# Autodesk Inventor assembly: SolarPanel
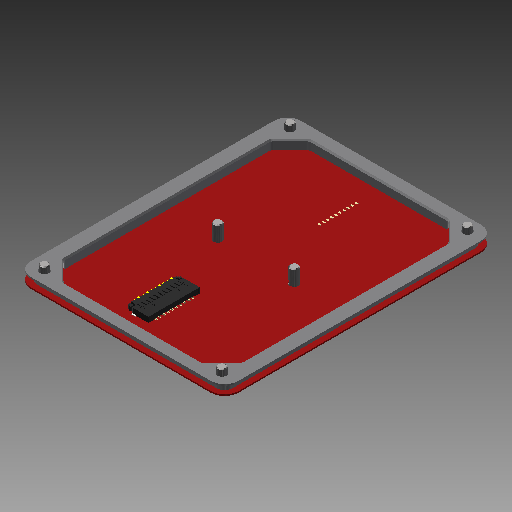
[picture p0: Inventor's stored thumbnail of the model, 512x512]
Saved by Autodesk Inventor 2018 (Build 220112000, 112)
## iProperties
Created: 2018-05-13
Part Number: SolarPanel
Document SubType Name: Assembly
Designer: Bradley
Mass: 16.4819 g
Surface Area: 334.424 cm^2
Volume: 10.2894 cm^3
Density: 1.60184 g/cm^3
Author: Bradley
## Documents named in this file (7)
- D:\Users\Bradley\Documents\CougsInSpace\CougSat1-Hardware\CougSat1-PowerBoard\CADModel\Native\SolarPanel+Y.iam
- D:\Users\Bradley\Documents\CougsInSpace\CougSat1-Hardware\CougSat1-PowerBoard\CADModel\Native\SolarPanel_PCB.ipt
- D:\Users\Bradley\Documents\CougsInSpace\CougSat1-Hardware\CougSat1-PowerBoard\CADModel\Native\SolarPanel_CoilForm.ipt
- D:\Users\Bradley\Documents\CougsInSpace\Resources\ComponentModels\Electronics\SolarCell_UTJ.ipt
- D:\Users\Bradley\Documents\CougsInSpace\Resources\ComponentModels\Fasteners\Bolt_M3x0.35_6mm_BH.ipt
- D:\Users\Bradley\Documents\CougsInSpace\Resources\ComponentModels\Connectors\PicoLock-J-10.ipt
- D:\Users\Bradley\Documents\CougsInSpace\Resources\ComponentModels\Connectors\PicoLock-P-10.ipt
## Components (12 placed, 6 different names)
1. SolarPanel_CoilForm:1 — Insert:1, Insert:2
2. SolarPanel_PCB:1 — Insert:1, Insert:2, Insert:3, Insert:4, Insert:5, Insert:6, Insert:7, Insert:8, Mate:1, Mate:2, Mate:7, Flush:4, Flush:5
3. PicoLock-J-10:1 — Mate:7, Flush:4, Flush:5
4. PicoLock-P-10:1
5. SolarCell_UTJ:1 — Mate:1, Flush:1, Flush:2
6. SolarCell_UTJ:2 — Mate:2, Mate:3, Mate:4
7. Bolt_M3x0.35_6mm_BH:1 — Insert:5
8. Bolt_M3x0.35_6mm_BH:2 — Insert:6
9. Bolt_M3x0.35_6mm_BH:6 — Insert:8
10. Bolt_M3x0.35_6mm_BH:7 — Insert:4
11. Bolt_M3x0.35_6mm_BH:8 — Insert:3
12. Bolt_M3x0.35_6mm_BH:5 — Insert:7
## Relationships (20: Insert 8, Mate 7, Flush 5)
- Insert:1: SolarPanel_CoilForm:1 ↔ SolarPanel_PCB:1
- Insert:2: SolarPanel_CoilForm:1 ↔ SolarPanel_PCB:1
- Insert:3: SolarPanel_PCB:1 ↔ Bolt_M3x0.35_6mm_BH:8
- Insert:4: SolarPanel_PCB:1 ↔ Bolt_M3x0.35_6mm_BH:7
- Insert:5: SolarPanel_PCB:1 ↔ Bolt_M3x0.35_6mm_BH:1
- Insert:6: SolarPanel_PCB:1 ↔ Bolt_M3x0.35_6mm_BH:2
- Insert:7: SolarPanel_PCB:1 ↔ Bolt_M3x0.35_6mm_BH:5
- Insert:8: SolarPanel_PCB:1 ↔ Bolt_M3x0.35_6mm_BH:6
- Mate:1: SolarPanel_PCB:1 ↔ SolarCell_UTJ:1
- Mate:2: SolarPanel_PCB:1 ↔ SolarCell_UTJ:2
- Flush:1: SolarCell_UTJ:1
- Mate:3: SolarCell_UTJ:2
- Mate:4 (5 mm): SolarCell_UTJ:2
- Flush:2 (5 mm): SolarCell_UTJ:1
- [Mate] (0.025 mm): PicoLock-J-10:1 ↔ PicoLock-P-10:1
- [Mate]: PicoLock-J-10:1 ↔ PicoLock-P-10:1
- [Flush]: PicoLock-J-10:1 ↔ PicoLock-P-10:1
- Mate:7: SolarPanel_PCB:1 ↔ PicoLock-J-10:1
- Flush:4 (0.15 mm): SolarPanel_PCB:1 ↔ PicoLock-J-10:1
- Flush:5 (-0.15 mm): SolarPanel_PCB:1 ↔ PicoLock-J-10:1
